# Autodesk Inventor assembly: levantador
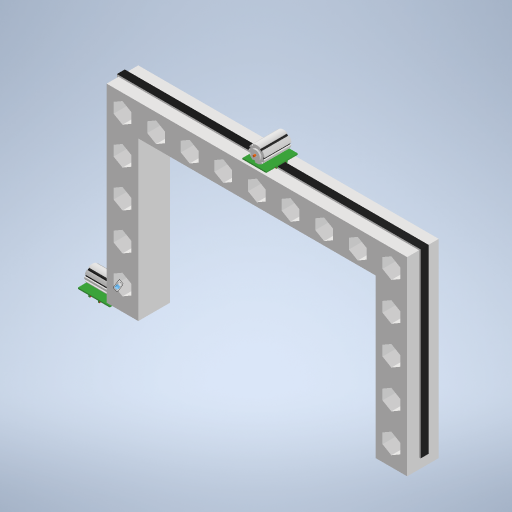
[picture p0: Inventor's stored thumbnail of the model, 512x512]
Saved by Autodesk Inventor 2023 (Build 270158000, 158)
## iProperties
Created: 2022-04-04
Part Number: levantador
Document SubType Name: Assembly
Designer: isaac
Author: isaac
## Documents named in this file (3)
- C:\Users\isaac\OneDrive\Documentos\Diseño mecánico\levantador.iam
- C:\Users\isaac\OneDrive\Documentos\Diseño mecánico\motor.ipt
- C:\Users\isaac\OneDrive\Documentos\Diseño mecánico\estructura.ipt
## Components (3 placed, 2 different names)
1. motor:1 — Corredera:1
2. motor:2 — Rígido:1
3. estructura:1 — Corredera:1, Rígido:1
## Relationships (2: TranslationJoint 1, WeldJoint 1)
- Corredera:1 [TranslationJoint]: motor:1 ↔ estructura:1
- Rígido:1 [WeldJoint]: motor:2 ↔ estructura:1
